# Autodesk Inventor assembly: Base
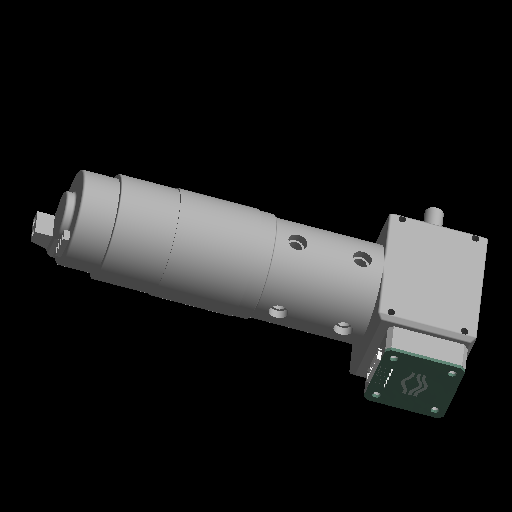
[picture p0: Inventor's stored thumbnail of the model, 512x512]
Saved by Autodesk Inventor 2025.2 (Build 292293000, 293)
## iProperties
Created: 2020-03-24
Part Number: Base
Document SubType Name: Assembly
Designer: valer
Mass: 715.256 g
Surface Area: 821.775 cm^2
Volume: 200.817 cm^3
Density: 3.56173 g/cm^3
Author: valer
## Documents named in this file (7)
- C:\Users\valer\Desktop\str1ker\cad\ArmBase.iam
- C:\Users\valer\Desktop\str1ker\cad\external\ShoulderActuator\DumaDynamics00E.ipt
- C:\Users\valer\Desktop\str1ker\cad\ShoulderEncoderSpacer.ipt
- C:\Users\valer\Desktop\str1ker\cad\external\ArmEncoder\ArmEncoderShaftMagnet6mm.ipt
- C:\Users\valer\Desktop\str1ker\cad\ShoulderEncoderFlange.ipt
- C:\Users\valer\Desktop\str1ker\cad\BaseBoundingBox.ipt
- C:\Users\valer\Desktop\str1ker\cad\external\ArmEncoder\ArmEncoderBoard.iam
## Components (6 placed, 6 different names)
1. DumaDynamics00E:1 — Flush:1, Mate:16, Mate:17, Flush:5, Mate:39, Mate:44, Mate:45, Mate:46
2. ArmEncoderShaftMagnet6mm:1 — Mate:16, Mate:17, Mate:25, Flush:4
3. ShoulderEncoderFlange:1 — Mate:25, Flush:4
4. BaseBoundingBox:1 — Mate:40
5. ArmEncoderBoard:1 [sub-assembly] — Mate:47, Mate:48, Mate:49
6. ShoulderEncoderSpacer:1 — Mate:44, Mate:45, Mate:46, Mate:47, Mate:48, Mate:49
## Relationships (14: Mate 11, Flush 3)
- Flush:1: DumaDynamics00E:1
- Mate:16: DumaDynamics00E:1 ↔ ArmEncoderShaftMagnet6mm:1
- Mate:17: DumaDynamics00E:1 ↔ ArmEncoderShaftMagnet6mm:1
- Mate:25: ArmEncoderShaftMagnet6mm:1 ↔ ShoulderEncoderFlange:1
- Flush:4: ArmEncoderShaftMagnet6mm:1 ↔ ShoulderEncoderFlange:1
- Flush:5 (6 mm): DumaDynamics00E:1
- Mate:39: DumaDynamics00E:1
- Mate:40: BaseBoundingBox:1
- Mate:44: DumaDynamics00E:1 ↔ ShoulderEncoderSpacer:1
- Mate:45: DumaDynamics00E:1 ↔ ShoulderEncoderSpacer:1
- Mate:46: DumaDynamics00E:1 ↔ ShoulderEncoderSpacer:1
- Mate:47: ArmEncoderBoard:1 ↔ ShoulderEncoderSpacer:1
- Mate:48: ArmEncoderBoard:1 ↔ ShoulderEncoderSpacer:1
- Mate:49: ArmEncoderBoard:1 ↔ ShoulderEncoderSpacer:1
